# Autodesk Inventor assembly: prototype1
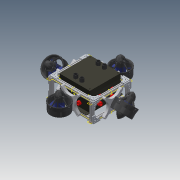
[picture p0: Inventor's stored thumbnail of the model, 180x180]
Saved by Autodesk Inventor 2018 (Build 220112000, 112)
## iProperties
Created: 2019-11-13
Part Number: prototype1
Document SubType Name: Assembly
Designer: anirudh
Author: anirudh
## Documents named in this file (7)
- C:\Users\anirudh\Documents\MARS Fund\MATE Robotics\Silicon Sharks\2019-2020\prototype1\prototype1.iam
- C:\Users\anirudh\Documents\MARS Fund\MATE Robotics\Silicon Sharks\2019-2020\ElectronicsHousing\Prototype2\ElectricalHousing2.iam
- C:\Users\anirudh\Documents\MARS Fund\MATE Robotics\Silicon Sharks\2019-2020\prototype1\8inREV.ipt
- C:\Users\anirudh\Documents\MARS Fund\MATE Robotics\Silicon Sharks\2019-2020\prototype1\3inREV.ipt
- C:\Users\anirudh\Documents\MARS Fund\Random CAD Files\REV-41-1480.ipt
- C:\Users\anirudh\Documents\MARS Fund\MATE Robotics\Silicon Sharks\2019-2020\prototype1\ThrusterMount.ipt
- C:\Users\anirudh\Documents\MARS Fund\MATE Robotics\Silicon Sharks\2019-2020\prototype1\T200-THRUSTER.ipt
## Components (37 placed, 6 different names)
1. ElectricalHousing2:1 [sub-assembly] — Mate:29, Flush:57, Mate:30
2. 8inREV:1 — Mate:1, Flush:1, Flush:2, Mate:2, Flush:3, Flush:4, Flush:7, Mate:6, Mate:7, Flush:13, Mate:8, Flush:15, Flush:16, Mate:9, Flush:17, Flush:18, Mate:27, Flush:49, Flush:52, Mate:40
3. 8inREV:2 — Mate:9, Flush:17, Flush:18, Mate:26, Flush:50, Flush:56, Mate:29, Flush:57, Mate:32, Mate:42
4. 8inREV:3 — Mate:8, Flush:15, Flush:16, Flush:25, Flush:26, Mate:13, Flush:51, Flush:54, Mate:38
5. 8inREV:4 — Mate:3, Flush:5, Flush:6, Mate:5, Flush:10, Flush:12, Mate:11, Mate:12, Flush:21, Flush:22, Flush:23, Mate:21, Mate:23, Flush:46, Flush:47, Mate:31, Mate:39, Mate:43
6. 8inREV:5 — Mate:12, Flush:22, Flush:23, Mate:14, Flush:27, Flush:28, Mate:24, Flush:43, Flush:45, Mate:34, Mate:37, Mate:44
7. 8inREV:6 — Mate:11, Flush:21, Flush:24, Mate:22, Flush:42, Flush:48, Mate:41, Mate:45
8. 8inREV:7 — Flush:25, Flush:26, Mate:13, Mate:15, Flush:29, Flush:30, Mate:16, Flush:31, Mate:17, Mate:19, Flush:34, Flush:40, Mate:25, Mate:28, Flush:53, Flush:55, Mate:30, Mate:33, Mate:36
9. 8inREV:8 — Mate:14, Flush:27, Flush:28, Flush:32, Mate:18, Mate:20, Flush:35, Flush:37, Flush:41, Flush:44, Mate:35, Mate:46
10. 3inREV:1 — Mate:1, Flush:1, Flush:2, Flush:11, Flush:14, Flush:24
11. 3inREV:2 — Mate:2, Flush:3, Flush:4, Mate:3, Flush:5, Flush:6, Mate:4, Flush:8, Flush:9
12. 3inREV:3 — Mate:15, Flush:29, Flush:30, Flush:38, Flush:39
13. 3inREV:4 — Mate:16, Flush:31, Flush:32, Flush:33, Flush:36
14. REV-41-1480:1 — Mate:7, Flush:13, Flush:14
15. REV-41-1480:2 — Mate:5, Flush:9, Flush:10
16. REV-41-1480:3 — Mate:4, Flush:7, Flush:8
17. REV-41-1480:4 — Mate:6, Flush:11, Flush:12
18. REV-41-1480:5 — Mate:19, Flush:39, Flush:40
19. REV-41-1480:6 — Mate:18, Flush:35, Flush:36
20. REV-41-1480:7 — Mate:28, Flush:53, Flush:54
21. REV-41-1480:8 — Mate:20, Flush:37, Flush:38
22. REV-41-1480:9 — Mate:25, Flush:55, Flush:56
23. REV-41-1480:10 — Mate:22, Flush:41, Flush:42
24. REV-41-1480:11 — Mate:24, Flush:43, Flush:44
25. REV-41-1480:12 — Mate:23, Flush:45, Flush:46
26. REV-41-1480:13 — Mate:21, Flush:47, Flush:48
27. REV-41-1480:14 — Mate:27, Flush:51, Flush:52
28. REV-41-1480:15 — Mate:26, Flush:49, Flush:50
29. REV-41-1480:16 — Mate:17, Flush:33, Flush:34
30. ThrusterMount:1 — Mate:31, Mate:39, Mate:40, Mate:43, Mate:61, Mate:62, Mate:63, Mate:64, Mate:65
31. ThrusterMount:2 — Mate:34, Mate:37, Mate:38, Mate:44, Mate:56, Mate:57, Mate:58, Mate:59, Mate:60
32. ThrusterMount:3 — Mate:33, Mate:35, Mate:36, Mate:46, Mate:66, Mate:67, Mate:68, Mate:69, Mate:70
33. ThrusterMount:4 — Mate:32, Mate:41, Mate:42, Mate:45, Mate:51, Mate:52, Mate:53, Mate:54, Mate:55
34. T200-THRUSTER:1 — Mate:61, Mate:62, Mate:63, Mate:64, Mate:65
35. T200-THRUSTER:2 — Mate:56, Mate:57, Mate:58, Mate:59, Mate:60
36. T200-THRUSTER:3 — Mate:66, Mate:67, Mate:68, Mate:69, Mate:70
37. T200-THRUSTER:4 — Mate:51, Mate:52, Mate:53, Mate:54, Mate:55
## Relationships (120: Mate 65, Flush 55)
- Mate:1: 8inREV:1 ↔ 3inREV:1
- Flush:1: 8inREV:1 ↔ 3inREV:1
- Flush:2: 8inREV:1 ↔ 3inREV:1
- Mate:2: 8inREV:1 ↔ 3inREV:2
- Flush:3: 8inREV:1 ↔ 3inREV:2
- Flush:4: 8inREV:1 ↔ 3inREV:2
- Mate:3: 8inREV:4 ↔ 3inREV:2
- Flush:5: 8inREV:4 ↔ 3inREV:2
- Flush:6: 8inREV:4 ↔ 3inREV:2
- Mate:4: 3inREV:2 ↔ REV-41-1480:3
- Flush:7: 8inREV:1 ↔ REV-41-1480:3
- Flush:8: 3inREV:2 ↔ REV-41-1480:3
- Mate:5: 8inREV:4 ↔ REV-41-1480:2
- Flush:9: 3inREV:2 ↔ REV-41-1480:2
- Flush:10: 8inREV:4 ↔ REV-41-1480:2
- Mate:6: 8inREV:1 ↔ REV-41-1480:4
- Flush:11: 3inREV:1 ↔ REV-41-1480:4
- Flush:12: 8inREV:4 ↔ REV-41-1480:4
- Mate:7: 8inREV:1 ↔ REV-41-1480:1
- Flush:13: 8inREV:1 ↔ REV-41-1480:1
- Flush:14: 3inREV:1 ↔ REV-41-1480:1
- Mate:8: 8inREV:1 ↔ 8inREV:3
- Flush:15 (4.4196 mm): 8inREV:1 ↔ 8inREV:3
- Flush:16: 8inREV:1 ↔ 8inREV:3
- Mate:9: 8inREV:1 ↔ 8inREV:2
- Flush:17: 8inREV:1 ↔ 8inREV:2
- Flush:18 (4.4196 mm): 8inREV:1 ↔ 8inREV:2
- Mate:11: 8inREV:4 ↔ 8inREV:6
- Mate:12: 8inREV:4 ↔ 8inREV:5
- Flush:21: 8inREV:4 ↔ 8inREV:6
- Flush:22: 8inREV:4 ↔ 8inREV:5
- Flush:23 (4.4196 mm): 8inREV:4 ↔ 8inREV:5
- Flush:24 (4.4196 mm): 8inREV:6 ↔ 3inREV:1
- Flush:25: 8inREV:3 ↔ 8inREV:7
- Flush:26: 8inREV:3 ↔ 8inREV:7
- Mate:13: 8inREV:3 ↔ 8inREV:7
- Mate:14: 8inREV:5 ↔ 8inREV:8
- Flush:27: 8inREV:5 ↔ 8inREV:8
- Flush:28: 8inREV:5 ↔ 8inREV:8
- Mate:15: 8inREV:7 ↔ 3inREV:3
- Flush:29: 8inREV:7 ↔ 3inREV:3
- Flush:30: 8inREV:7 ↔ 3inREV:3
- Mate:16: 8inREV:7 ↔ 3inREV:4
- Flush:31: 8inREV:7 ↔ 3inREV:4
- Flush:32: 8inREV:8 ↔ 3inREV:4
- Mate:17: 8inREV:7 ↔ REV-41-1480:16
- Mate:18: 8inREV:8 ↔ REV-41-1480:6
- Mate:19: 8inREV:7 ↔ REV-41-1480:5
- Mate:20: 8inREV:8 ↔ REV-41-1480:8
- Flush:33: 3inREV:4 ↔ REV-41-1480:16
- Flush:34: 8inREV:7 ↔ REV-41-1480:16
- Flush:35: 8inREV:8 ↔ REV-41-1480:6
- Flush:36: 3inREV:4 ↔ REV-41-1480:6
- Flush:37: 8inREV:8 ↔ REV-41-1480:8
- Flush:38: 3inREV:3 ↔ REV-41-1480:8
- Flush:39: 3inREV:3 ↔ REV-41-1480:5
- Flush:40: 8inREV:7 ↔ REV-41-1480:5
- Mate:21: 8inREV:4 ↔ REV-41-1480:13
- Mate:22: 8inREV:6 ↔ REV-41-1480:10
- Mate:23: 8inREV:4 ↔ REV-41-1480:12
- Mate:24: 8inREV:5 ↔ REV-41-1480:11
- Flush:41: 8inREV:8 ↔ REV-41-1480:10
- Flush:42: 8inREV:6 ↔ REV-41-1480:10
- Flush:43: 8inREV:5 ↔ REV-41-1480:11
- Flush:44: 8inREV:8 ↔ REV-41-1480:11
- Flush:45: 8inREV:5 ↔ REV-41-1480:12
- Flush:46: 8inREV:4 ↔ REV-41-1480:12
- Flush:47: 8inREV:4 ↔ REV-41-1480:13
- Flush:48: 8inREV:6 ↔ REV-41-1480:13
- Mate:25: 8inREV:7 ↔ REV-41-1480:9
- Mate:26: 8inREV:2 ↔ REV-41-1480:15
- Mate:27: 8inREV:1 ↔ REV-41-1480:14
- Mate:28: 8inREV:7 ↔ REV-41-1480:7
- Flush:49: 8inREV:1 ↔ REV-41-1480:15
- Flush:50: 8inREV:2 ↔ REV-41-1480:15
- Flush:51: 8inREV:3 ↔ REV-41-1480:14
- Flush:52: 8inREV:1 ↔ REV-41-1480:14
- Flush:53: 8inREV:7 ↔ REV-41-1480:7
- Flush:54: 8inREV:3 ↔ REV-41-1480:7
- Flush:55: 8inREV:7 ↔ REV-41-1480:9
- Flush:56: 8inREV:2 ↔ REV-41-1480:9
- Mate:29: ElectricalHousing2:1 ↔ 8inREV:2
- Flush:57: ElectricalHousing2:1 ↔ 8inREV:2
- Mate:30 (-38.0238 mm): ElectricalHousing2:1 ↔ 8inREV:7
- Mate:31: 8inREV:4 ↔ ThrusterMount:1
- Mate:32: 8inREV:2 ↔ ThrusterMount:4
- Mate:33: 8inREV:7 ↔ ThrusterMount:3
- Mate:34: 8inREV:5 ↔ ThrusterMount:2
- Mate:35: 8inREV:8 ↔ ThrusterMount:3
- Mate:36: 8inREV:7 ↔ ThrusterMount:3
- Mate:37: 8inREV:5 ↔ ThrusterMount:2
- Mate:38: 8inREV:3 ↔ ThrusterMount:2
- Mate:39: 8inREV:4 ↔ ThrusterMount:1
- Mate:40: 8inREV:1 ↔ ThrusterMount:1
- Mate:41: 8inREV:6 ↔ ThrusterMount:4
- Mate:42: 8inREV:2 ↔ ThrusterMount:4
- Mate:43: 8inREV:4 ↔ ThrusterMount:1
- Mate:44: 8inREV:5 ↔ ThrusterMount:2
- Mate:45: 8inREV:6 ↔ ThrusterMount:4
- Mate:46: 8inREV:8 ↔ ThrusterMount:3
- Mate:51: ThrusterMount:4 ↔ T200-THRUSTER:4
- Mate:52: ThrusterMount:4 ↔ T200-THRUSTER:4
- Mate:53: ThrusterMount:4 ↔ T200-THRUSTER:4
- Mate:54: ThrusterMount:4 ↔ T200-THRUSTER:4
- Mate:55: ThrusterMount:4 ↔ T200-THRUSTER:4
- Mate:56: ThrusterMount:2 ↔ T200-THRUSTER:2
- Mate:57: ThrusterMount:2 ↔ T200-THRUSTER:2
- Mate:58: ThrusterMount:2 ↔ T200-THRUSTER:2
- Mate:59: ThrusterMount:2 ↔ T200-THRUSTER:2
- Mate:60: ThrusterMount:2 ↔ T200-THRUSTER:2
- Mate:61: ThrusterMount:1 ↔ T200-THRUSTER:1
- Mate:62: ThrusterMount:1 ↔ T200-THRUSTER:1
- Mate:63: ThrusterMount:1 ↔ T200-THRUSTER:1
- Mate:64: ThrusterMount:1 ↔ T200-THRUSTER:1
- Mate:65: ThrusterMount:1 ↔ T200-THRUSTER:1
- Mate:66: ThrusterMount:3 ↔ T200-THRUSTER:3
- Mate:67: ThrusterMount:3 ↔ T200-THRUSTER:3
- Mate:68: ThrusterMount:3 ↔ T200-THRUSTER:3
- Mate:69: ThrusterMount:3 ↔ T200-THRUSTER:3
- Mate:70: ThrusterMount:3 ↔ T200-THRUSTER:3
